# Autodesk Inventor assembly: Power
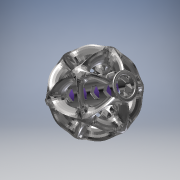
[picture p0: Inventor's stored thumbnail of the model, 180x180]
Saved by Autodesk Inventor 2019 (Build 230136000, 136)
## iProperties
Created: 2019-05-09
Part Number: Power
Document SubType Name: Assembly
Designer: Jorian Brusind
Author: Jorian Brusind
## Documents named in this file (3)
- C:\Users\Jorian Brusind\Documents\GitHub\PersonalProjects\Inventor Projects\Infinity\Power.iam
- C:\Users\Jorian Brusind\Documents\GitHub\PersonalProjects\Inventor Projects\Infinity\Purple.ipt
- C:\Users\Jorian Brusind\Documents\GitHub\PersonalProjects\Inventor Projects\Infinity\Orb.ipt
## Components (2 placed, 2 different names)
1. Purple:1 — Mate:1, Mate:2
2. Orb:1 — Mate:1, Mate:2
## Relationships (2: Mate 2)
- Mate:1: Purple:1 ↔ Orb:1
- Mate:2: Purple:1 ↔ Orb:1
## Named parameters: sa_0 = 6894.76
note: some values were not read from the file. Shown as the stored number, unit unknown: "sa_0".
